# Autodesk Inventor assembly: FGS
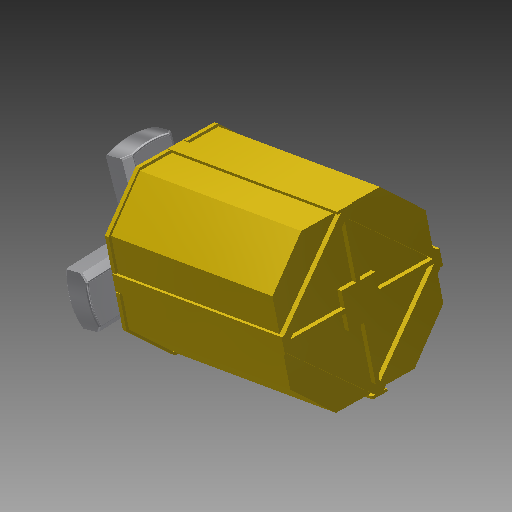
[picture p0: Inventor's stored thumbnail of the model, 512x512]
Saved by Autodesk Inventor 2018 (Build 220112000, 112)
## iProperties
Created: 2021-03-14
Part Number: FGS
Document SubType Name: Assembly
Designer: NITESH MAURYA
Author: NITESH MAURYA
## Documents named in this file (4)
- C:\Users\dell\Desktop\ES101 GROUP-13 PROJECT\FINAL MODEL\Resolved files\Assembly1.iam
- C:\Users\dell\Desktop\ES101 GROUP-13 PROJECT\INDIVIDUAL WORK\Nitesh\Resolved Parts\Derived FGS.ipt
- C:\Users\dell\Desktop\ES101 GROUP-13 PROJECT\INDIVIDUAL WORK\Nitesh\SupportingRod_CPY.ipt
- C:\Users\dell\Desktop\ES101 GROUP-13 PROJECT\INDIVIDUAL WORK\Tejas\Part1 - Instrument modules.ipt
## Components (7 placed, 3 different names)
1. Derived FGS:1 — Mate:3, Mate:7
2. Derived FGS:2 — Mate:3, Mate:4, Mate:12
3. Derived FGS:3 — Mate:4, Mate:6
4. SupportingRod_CPY:2 — Mate:6, Mate:9
5. SupportingRod_CPY:3 — Mate:7, Mate:10
6. Part1 - Instrument modules:1 — Mate:9, Mate:10
7. SupportingRod_CPY:4 — Mate:12
## Relationships (7: Mate 7)
- Mate:3 (12.7 mm): Derived FGS:1 ↔ Derived FGS:2
- Mate:4 (12.7 mm): Derived FGS:2 ↔ Derived FGS:3
- Mate:6: Derived FGS:3 ↔ SupportingRod_CPY:2
- Mate:7: Derived FGS:1 ↔ SupportingRod_CPY:3
- Mate:9: SupportingRod_CPY:2 ↔ Part1 - Instrument modules:1
- Mate:10: SupportingRod_CPY:3 ↔ Part1 - Instrument modules:1
- Mate:12: Derived FGS:2 ↔ SupportingRod_CPY:4
